# Autodesk Inventor assembly: M178-PHTM-FLC-LCD-1600x1200-17
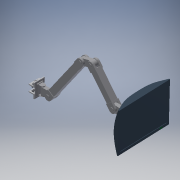
[picture p0: Inventor's stored thumbnail of the model, 180x180]
Saved by Autodesk Inventor 2018 (Build 220105000, 105)
## iProperties
Created: 2004-11-29
Part Number: M178-PHTM-FLC-LCD-1600x1200-17
Document SubType Name: Assembly
Designer: Autodesk, Inc.
Manufacturer: Standard
Standards Organization: Custom
Mass: 6597.31 g
Surface Area: 5882.76 cm^2
Volume: 6416.93 cm^3
Density: 1.02811 g/cm^3
CAGE: 1LJX3
Dept. ID: Product Design
Description #2: ---
Finish #1: ---
Finish #2: ---
Material ID: ---
Project Number: ---
Author: Autodesk, Inc.
## Documents named in this file (11)
- C:\Autodesk\autodesk_inventor_2017_samples\Models\Assemblies\Test Station\Components\Monitor Phantom.iam
- C:\Autodesk\autodesk_inventor_2017_samples\Models\Assemblies\Test Station\Components\FLC-LCD-1600x1200-17.ipt
- C:\Autodesk\autodesk_inventor_2017_samples\Models\Assemblies\Test Station\Components\SwingArm.iam
- C:\Autodesk\autodesk_inventor_2017_samples\Models\Assemblies\Test Station\Components\Monitor Arm Ref Cross Bar.ipt
- C:\Autodesk\autodesk_inventor_2017_samples\Models\Assemblies\Test Station\Components\M178-3502.ipt
- C:\Autodesk\autodesk_inventor_2017_samples\Models\Assemblies\Test Station\Components\24-112-8.ipt
- C:\Autodesk\autodesk_inventor_2017_samples\Models\Assemblies\Test Station\Components\20-058.ipt
- C:\Autodesk\autodesk_inventor_2017_samples\Models\Assemblies\Test Station\Components\24-18-5.ipt
- C:\Users\kelleyb.ADS\Desktop\Samples MIGRATED 2009 224 RTM_1\Standard Parts\Test Station Content\Extrusions\40 Series Profiles.ipt
- C:\Users\kelleyb.ADS\Desktop\Samples MIGRATED 2009 224 RTM_1\Standard Parts\Test Station Content\Fastners\2X-YYY-ZZ IPS Screws.ipt
- C:\Users\kelleyb.ADS\Desktop\Samples MIGRATED 2009 224 RTM_1\Standard Parts\Test Station Content\Fastners\20-XXX TSlot Nuts.ipt
## Components (17 placed, 7 different names)
1. FLC-LCD-1600x1200-17:1
2. SwingArm:1 [sub-assembly] — Mate:1, Flush:1, Mate:2, Mate:4, Insert:3, Insert:4, Mate:12, Insert:9, Insert:10
3. Monitor Arm Ref Cross Bar:1 — Mate:1, Mate:3, Mate:11
4. M178-3502:1 — Flush:2, Mate:3, Mate:4, Insert:5, Insert:6, Mate:7, Angle:1, Angle:2
5. 24-112-8:1 — Insert:6, Mate:5
6. 24-112-8:2 — Insert:5, Mate:6
7. 24-18-5:5 — Insert:4
8. 24-18-5:6 — Insert:3
9. 20-058:1 — Mate:5, Mate:7, Flush:3, Angle:1
10. 20-058:2 — Mate:6, Flush:3, Angle:2
11. M178-3502:2 — Flush:4, Insert:7, Insert:8, Angle:3, Angle:4, Mate:8, Mate:11, Mate:12
12. 24-112-8:3 — Insert:7, Mate:10
13. 24-112-8:4 — Insert:8, Mate:9
14. 24-18-5:7 — Insert:10
15. 24-18-5:8 — Insert:9
16. 20-058:3 — Angle:4, Flush:5, Mate:8, Mate:10
17. 20-058:4 — Angle:3, Flush:5, Mate:9
## Relationships (31: Mate 12, Insert 10, Flush 5, Angle 4)
- [Insert]: FLC-LCD-1600x1200-17:1 ↔ SwingArm:1
- [Insert]: FLC-LCD-1600x1200-17:1 ↔ SwingArm:1
- Mate:1: SwingArm:1 ↔ Monitor Arm Ref Cross Bar:1
- Flush:1: SwingArm:1
- Mate:2: SwingArm:1
- Flush:2: M178-3502:1
- Mate:3: Monitor Arm Ref Cross Bar:1 ↔ M178-3502:1
- Mate:4: SwingArm:1 ↔ M178-3502:1
- Insert:3: SwingArm:1 ↔ 24-18-5:6
- Insert:4: SwingArm:1 ↔ 24-18-5:5
- Insert:5: M178-3502:1 ↔ 24-112-8:2
- Insert:6: M178-3502:1 ↔ 24-112-8:1
- Mate:5: 24-112-8:1 ↔ 20-058:1
- Mate:6: 24-112-8:2 ↔ 20-058:2
- Mate:7 (4.5 mm): M178-3502:1 ↔ 20-058:1
- Flush:3: 20-058:1 ↔ 20-058:2
- Angle:1 (0 deg): M178-3502:1 ↔ 20-058:1
- Angle:2 (0 deg): M178-3502:1 ↔ 20-058:2
- Flush:4: M178-3502:2
- Insert:7: M178-3502:2 ↔ 24-112-8:3
- Insert:8: M178-3502:2 ↔ 24-112-8:4
- Angle:3 (0 deg): M178-3502:2 ↔ 20-058:4
- Angle:4 (0 deg): M178-3502:2 ↔ 20-058:3
- Flush:5: 20-058:3 ↔ 20-058:4
- Mate:8 (4.5 mm): M178-3502:2 ↔ 20-058:3
- Mate:9: 24-112-8:4 ↔ 20-058:4
- Mate:10: 24-112-8:3 ↔ 20-058:3
- Mate:11: Monitor Arm Ref Cross Bar:1 ↔ M178-3502:2
- Mate:12: SwingArm:1 ↔ M178-3502:2
- Insert:9: SwingArm:1 ↔ 24-18-5:8
- Insert:10: SwingArm:1 ↔ 24-18-5:7
